# Autodesk Inventor assembly: panel assembly
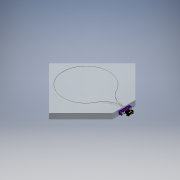
[picture p0: Inventor's stored thumbnail of the model, 180x180]
Saved by Autodesk Inventor 2016 (Build 200138000, 138)
## iProperties
Created: 2016-08-11
Part Number: panel assembly
Document SubType Name: Assembly
Designer: Jonathan
Author: Jonathan
## Documents named in this file (4)
- C:\Users\Jonathan\Documents\Projects\muonTelescope\panel assembly\panel assembly.iam
- C:\Users\Jonathan\Documents\Projects\muonTelescope\dependency\scintillatorPanel\loopPanel.iam
- C:\Users\Jonathan\Documents\Projects\muonTelescope\dependency\mppcSensor\cad\mppcSensor.iam
- C:\Users\Jonathan\Documents\Projects\muonTelescope\panel assembly\4-40 half inch screw.ipt
## Components (4 placed, 3 different names)
1. loopPanel:1 [sub-assembly] — Mate:1, Mate:2, Mate:3
2. mppcSensor:1 [sub-assembly] — Mate:1, Mate:2, Mate:3, Mate:4, Mate:5, Mate:6, Mate:7, Angle:1, Angle:2
3. 4-40 half inch screw:1 — Mate:4, Mate:6, Angle:1
4. 4-40 half inch screw:2 — Mate:5, Mate:7, Angle:2
## Relationships (9: Mate 7, Angle 2)
- Mate:1: loopPanel:1 ↔ mppcSensor:1
- Mate:2: loopPanel:1 ↔ mppcSensor:1
- Mate:3: loopPanel:1 ↔ mppcSensor:1
- Mate:4: mppcSensor:1 ↔ 4-40 half inch screw:1
- Mate:5: mppcSensor:1 ↔ 4-40 half inch screw:2
- Mate:6: mppcSensor:1 ↔ 4-40 half inch screw:1
- Mate:7: mppcSensor:1 ↔ 4-40 half inch screw:2
- Angle:1 (0 deg): mppcSensor:1 ↔ 4-40 half inch screw:1
- Angle:2 (0 deg): mppcSensor:1 ↔ 4-40 half inch screw:2
